# Autodesk Inventor assembly: dribbler_v2
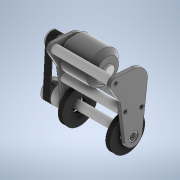
[picture p0: Inventor's stored thumbnail of the model, 180x180]
Saved by Autodesk Inventor 2020 (Build 240168000, 168)
## iProperties
Created: 2024-02-24
Part Number: dribbler_v2
Document SubType Name: Assembly
Designer: 4s
Author: 4s
## Documents named in this file (10)
- C:\Users\4s\Documents\Inventor models\Asterisk\robot_v2\dribbler\dribbler_v2.iam
- C:\Users\4s\Documents\Inventor models\Asterisk\robot_v2\dribbler\right_wall_v1.ipt
- C:\Users\4s\Documents\Inventor models\Asterisk\robot_v2\dribbler\motor_sketch.ipt
- C:\Users\4s\Documents\Inventor models\Asterisk\robot_v2\dribbler\roller_5_8_25.ipt
- C:\Users\4s\Documents\Inventor models\Asterisk\robot_v2\dribbler\left_wall_v1.ipt
- C:\Users\4s\Documents\Inventor models\Asterisk\robot_v2\dribbler\gear_16.ipt
- C:\Users\4s\Documents\Inventor models\Asterisk\robot_v2\dribbler\gear_20.ipt
- C:\Users\4s\Documents\Inventor models\Asterisk\robot_v2\dribbler\wheel.ipt
- C:\Users\4s\Documents\Inventor models\Asterisk\robot_v2\dribbler\stand_50.ipt
- C:\Users\4s\Documents\Inventor models\Asterisk\robot_v2\dribbler\remen.ipt
## Components (14 placed, 9 different names)
1. right_wall_v1:1 — Совмещение:1, Совмещение:2, Совмещение:3, Совмещение:7, Заподлицо:1, Совмещение:8, Совмещение:9, Совмещение:12, Совмещение:14, Совмещение:18, Совмещение:19, Совмещение:20, Симметрия:1, Совмещение:22, Совмещение:25, Совмещение:30, Совмещение:31, Совмещение:33
2. roller_5_8_25:1 — Совмещение:7, Заподлицо:1, Совмещение:13, Совмещение:15
3. left_wall_v1:1 — Совмещение:8, Совмещение:9, Совмещение:10, Заподлицо:2, Совмещение:17, Совмещение:19, Совмещение:21, Симметрия:1, Совмещение:23, Совмещение:26, Совмещение:27
4. roller_5_8_25:2 — Совмещение:10, Заподлицо:2, Совмещение:16, Совмещение:24
5. gear_16:1 — Совмещение:12, ЗубчПер:1, Совмещение:32
6. gear_20:1 — Совмещение:13, Совмещение:14, ЗубчПер:1, Совмещение:28, Совмещение:29
7. wheel:1 — Совмещение:16, Совмещение:17
8. wheel:2 — Совмещение:15, Совмещение:18
9. stand_50:1 — Совмещение:20, Совмещение:21
10. stand_50:2 — Совмещение:22, Совмещение:23
11. stand_50:3 — Совмещение:24, Совмещение:25
12. stand_50:4 — Совмещение:26, Совмещение:27
13. remen:1 — Совмещение:28, Совмещение:29
14. motor_sketch:2 — Совмещение:30, Совмещение:31, Совмещение:32, Совмещение:33
## Relationships (33: Mate 29, Flush 2, Symmetry 1, RelateRotation 1)
- Совмещение:1 [Mate]: right_wall_v1:1
- Совмещение:2 [Mate]: right_wall_v1:1
- Совмещение:3 [Mate]: right_wall_v1:1
- Совмещение:7 [Mate]: right_wall_v1:1 ↔ roller_5_8_25:1
- Заподлицо:1 [Flush] (0.25 mm): right_wall_v1:1 ↔ roller_5_8_25:1
- Совмещение:8 [Mate]: right_wall_v1:1 ↔ left_wall_v1:1
- Совмещение:9 [Mate]: right_wall_v1:1 ↔ left_wall_v1:1
- Совмещение:10 [Mate]: left_wall_v1:1 ↔ roller_5_8_25:2
- Заподлицо:2 [Flush] (0.25 mm): left_wall_v1:1 ↔ roller_5_8_25:2
- Совмещение:12 [Mate] (2 mm): right_wall_v1:1 ↔ gear_16:1
- Совмещение:13 [Mate]: roller_5_8_25:1 ↔ gear_20:1
- Совмещение:14 [Mate] (1 mm): right_wall_v1:1 ↔ gear_20:1
- Совмещение:15 [Mate]: roller_5_8_25:1 ↔ wheel:2
- Совмещение:16 [Mate]: roller_5_8_25:2 ↔ wheel:1
- Совмещение:17 [Mate] (3 mm): left_wall_v1:1 ↔ wheel:1
- Совмещение:18 [Mate] (3 mm): right_wall_v1:1 ↔ wheel:2
- Совмещение:19 [Mate] (50 mm): right_wall_v1:1 ↔ left_wall_v1:1
- Совмещение:20 [Mate]: right_wall_v1:1 ↔ stand_50:1
- Совмещение:21 [Mate]: left_wall_v1:1 ↔ stand_50:1
- Симметрия:1 [Symmetry]: right_wall_v1:1 ↔ left_wall_v1:1
- Совмещение:22 [Mate]: right_wall_v1:1 ↔ stand_50:2
- Совмещение:23 [Mate]: left_wall_v1:1 ↔ stand_50:2
- ЗубчПер:1 [RelateRotation] (1.25 ul): gear_16:1 ↔ gear_20:1
- Совмещение:24 [Mate]: roller_5_8_25:2 ↔ stand_50:3
- Совмещение:25 [Mate]: right_wall_v1:1 ↔ stand_50:3
- Совмещение:26 [Mate]: left_wall_v1:1 ↔ stand_50:4
- Совмещение:27 [Mate]: left_wall_v1:1 ↔ stand_50:4
- Совмещение:28 [Mate]: gear_20:1 ↔ remen:1
- Совмещение:29 [Mate] (0.5 mm): gear_20:1 ↔ remen:1
- Совмещение:30 [Mate]: right_wall_v1:1 ↔ motor_sketch:2
- Совмещение:31 [Mate]: right_wall_v1:1 ↔ motor_sketch:2
- Совмещение:32 [Mate]: gear_16:1 ↔ motor_sketch:2
- Совмещение:33 [Mate]: right_wall_v1:1 ↔ motor_sketch:2
